# Autodesk Inventor assembly: A_Flightcontroller_PCB
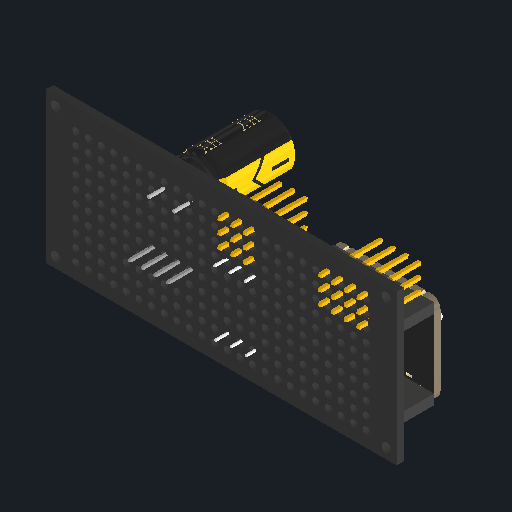
[picture p0: Inventor's stored thumbnail of the model, 512x512]
Saved by Autodesk Inventor 2026 (Build 300175000, 175)
## iProperties
Created: 2025-09-06
Part Number: A_Flightcontroller_PCB
Document SubType Name: Assembly
Designer: FAL
Author: FAL
## Documents named in this file (9)
- C:\Users\FAL\Projekte\Git\AIRBERT\CAD\Electronic\Flightcontroller_PCB\A_Flightcontroller_PCB.iam
- C:\Users\FAL\Projekte\Git\AIRBERT\CAD\Electronic\Flightcontroller_PCB\P_PCB_40x60.ipt
- C:\Users\FAL\Projekte\Git\AIRBERT\CAD\Electronic\Flightcontroller_PCB\PinHeader\Pin Header 1x3 TH Pitch 2.54mm\Pin Header 1x3 TH Pitch 2.54mm\Pin Header 1x3 TH Pitch 2.54mm.ipt
- C:\Users\FAL\Projekte\Git\AIRBERT\CAD\Electronic\Flightcontroller_PCB\PinHeader\Pin Header 1x3 TH Pitch 2.54mm\AHT20+BMP280\AHT20+BMP280.ipt
- C:\Users\FAL\Projekte\Git\AIRBERT\CAD\Electronic\Flightcontroller_PCB\PinHeader\Pin Header 1x3 TH Pitch 2.54mm\MPU6050 Accelerometer\MPU6050 Accelerometer.ipt
- C:\Users\FAL\Projekte\Git\AIRBERT\CAD\Electronic\Flightcontroller_PCB\XIAO-ESP32S3 v2.iam
- C:\Users\FAL\Projekte\Git\AIRBERT\CAD\Electronic\Flightcontroller_PCB\P_Spacer_Dummy_ESP32C3.ipt
- C:\Users\FAL\Projekte\Git\AIRBERT\CAD\Electronic\Flightcontroller_PCB\resistors\Resistor Axial 0.5W - Pitch 12.7mm (500mil) - Value 270R\Resistor Axial 0.5W - Pitch 12.7mm (500mil) - Value 270R\Resistor Axial 0.ipt
- C:\Users\FAL\Projekte\Git\AIRBERT\CAD\Electronic\Flightcontroller_PCB\Electrolytic capacitors\El_5_10_17._Black\El_5_10_17._Black\El_5_10_17._Black.ipt
## Components (17 placed, 8 different names)
1. P_PCB_40x60:1 — Fluchtend:1, Fluchtend:2, Fluchtend:5, Fluchtend:6, Fluchtend:7, Passend:12, Passend:13, Passend:18
2. Pin Header 1x3 TH Pitch 2.54mm:1
3. Pin Header 1x3 TH Pitch 2.54mm:2
4. Pin Header 1x3 TH Pitch 2.54mm:3
5. Pin Header 1x3 TH Pitch 2.54mm:4
6. AHT20+BMP280:1 — Passend:12
7. MPU6050 Accelerometer:1 — Passend:13
8. XIAO-ESP32S3 v2:1 [sub-assembly] — Fluchtend:16, Fluchtend:17, Passend:16, Passend:17, Fluchtend:20
9. P_Spacer_Dummy_ESP32C3:1 — Fluchtend:16, Fluchtend:17, Passend:16, Fluchtend:19, Passend:18
10. P_Spacer_Dummy_ESP32C3:2 — Fluchtend:19, Passend:17, Fluchtend:20
11. Pin Header 1x3 TH Pitch 2.54mm:9
12. Pin Header 1x3 TH Pitch 2.54mm:10
13. Pin Header 1x3 TH Pitch 2.54mm:12
14. Resistor Axial 0:1
15. Resistor Axial 0:2
16. Resistor Axial 0:3
17. El_5_10_17._Black:1
## Relationships (14: Flush 9, Mate 5)
- Fluchtend:1 [Flush]: P_PCB_40x60:1
- Fluchtend:2 [Flush]: P_PCB_40x60:1
- Fluchtend:5 [Flush]: P_PCB_40x60:1
- Fluchtend:6 [Flush]: P_PCB_40x60:1
- Fluchtend:7 [Flush]: P_PCB_40x60:1
- Passend:12 [Mate]: P_PCB_40x60:1 ↔ AHT20+BMP280:1
- Passend:13 [Mate]: P_PCB_40x60:1 ↔ MPU6050 Accelerometer:1
- Fluchtend:16 [Flush]: XIAO-ESP32S3 v2:1 ↔ P_Spacer_Dummy_ESP32C3:1
- Fluchtend:17 [Flush]: XIAO-ESP32S3 v2:1 ↔ P_Spacer_Dummy_ESP32C3:1
- Passend:16 [Mate]: XIAO-ESP32S3 v2:1 ↔ P_Spacer_Dummy_ESP32C3:1
- Fluchtend:19 [Flush]: P_Spacer_Dummy_ESP32C3:1 ↔ P_Spacer_Dummy_ESP32C3:2
- Passend:17 [Mate]: XIAO-ESP32S3 v2:1 ↔ P_Spacer_Dummy_ESP32C3:2
- Fluchtend:20 [Flush]: XIAO-ESP32S3 v2:1 ↔ P_Spacer_Dummy_ESP32C3:2
- Passend:18 [Mate]: P_PCB_40x60:1 ↔ P_Spacer_Dummy_ESP32C3:1
